(part 1 of 2)
# Autodesk Inventor assembly: Intake Full Assembly
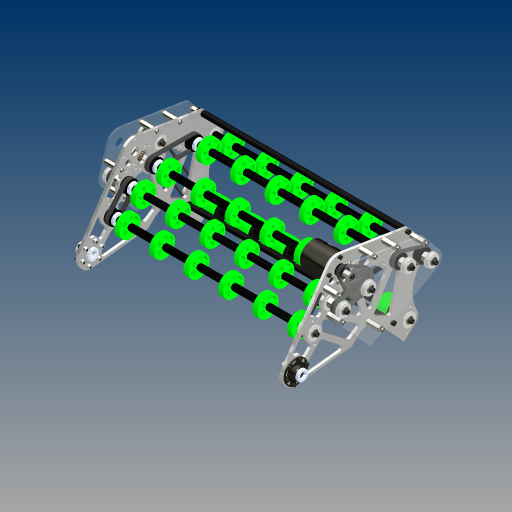
[picture p0: Inventor's stored thumbnail of the model, 512x512]
Saved by Autodesk Inventor 2024.3 (Build 283343000, 343)
## iProperties
Created: 2024-07-29
Part Number: Intake Full Assembly
Document SubType Name: Assembly
Designer: Kenji
Mass: 5624.47 g
Surface Area: 12461.9 cm^2
Volume: 2500.15 cm^3
Density: 2.24965 g/cm^3
Author: Kenji
## Documents named in this file (37)
- C:\Users\Kenji\Documents\GitHub\1622-2024-Summer-CAD-A-Thon\Intake\Intake Full Assembly.iam
- C:\Users\Kenji\Documents\GitHub\1622-2024-Summer-CAD-A-Thon\Intake\Intake Roller Plate.ipt
- C:\Users\Kenji\Documents\GitHub\1622-2024-Summer-CAD-A-Thon\COTS Library\Motion\Bearings\COTS_WCP-0783_1.125ODHexBearing.ipt
- C:\Users\Kenji\Documents\GitHub\1622-2024-Summer-CAD-A-Thon\Intake\Intake HexShaft 1.ipt
- C:\Users\Kenji\Documents\GitHub\1622-2024-Summer-CAD-A-Thon\COTS Library\Motion\Wheels\Compliant Wheels\2in compliant wheels\0.500in hex bore\COTS_am-3462_2indiameter_0.500inhexbore_durometer35A_CompliantWheel.ipt
- C:\Users\Kenji\Documents\GitHub\1622-2024-Summer-CAD-A-Thon\COTS Library\Motion\Wheels\Stealth Wheels\COTS_am-3155 2IN 500Hex Stealth Wheel.iam
- C:\Users\Kenji\Documents\GitHub\1622-2024-Summer-CAD-A-Thon\COTS Library\Structural Adapter\VersaHubs\COTS_217-2592_VersaHub.ipt
- C:\Users\Kenji\Documents\GitHub\1622-2024-Summer-CAD-A-Thon\Intake\Intake BeaterBar.ipt
- C:\Users\Kenji\Documents\GitHub\1622-2024-Summer-CAD-A-Thon\COTS Library\Fasteners\Bolts\Socket-Head\0.25-20\COTS_91251A539_Black-Oxide Alloy Steel Socket Head Screw (1).ipt
- C:\Users\Kenji\Documents\GitHub\1622-2024-Summer-CAD-A-Thon\COTS Library\Fasteners\Washers\COTS_90107A029_316 Stainless Steel Washer.ipt
- C:\Users\Kenji\Documents\GitHub\1622-2024-Summer-CAD-A-Thon\COTS Library\Fasteners\Shaft Collars\COTS_WCP-0799_0.5inchHexShaftCollar.ipt
- C:\Users\Kenji\Documents\GitHub\1622-2024-Summer-CAD-A-Thon\COTS Library\Motors\COTS_REV-21-1650-V1.1.ipt
- C:\Users\Kenji\Documents\GitHub\1622-2024-Summer-CAD-A-Thon\Intake\Intake Hex Shaft 3.ipt
- C:\Users\Kenji\Documents\GitHub\1622-2024-Summer-CAD-A-Thon\COTS Library\Motion\Pulleys\HTD5M\10mm Wide\COTW_HTD5M10mm12T_WCP-0076.ipt
- C:\Users\Kenji\Documents\GitHub\1622-2024-Summer-CAD-A-Thon\COTS Library\Motion\Pulleys\HTD5M\10mm Wide\COTS_HTD5M10mm36T_WCP-0990.ipt
- C:\Users\Kenji\Documents\GitHub\1622-2024-Summer-CAD-A-Thon\COTS Library\Motion\Gears\20DP gears\Aluminum\COTS_WCP-0706_30T.ipt
- C:\Users\Kenji\Documents\GitHub\1622-2024-Summer-CAD-A-Thon\COTS Library\Motion\Pulleys\HTD5M\10mm Wide\COTS_HTD5M10mm18T_WCP-0563.ipt
- C:\Users\Kenji\Documents\GitHub\1622-2024-Summer-CAD-A-Thon\Intake\INTK_002_HexShaft4.ipt
- C:\Users\Kenji\Documents\GitHub\1622-2024-Summer-CAD-A-Thon\Intake\INTK_003_HexShaft5.ipt
- C:\Users\Kenji\Documents\GitHub\1622-2024-Summer-CAD-A-Thon\Intake\INTK_001_PulleyCover.ipt
- C:\Users\Kenji\Documents\GitHub\1622-2024-Summer-CAD-A-Thon\Intake\INTK_004_HexShaft6.ipt
- C:\Users\Kenji\Documents\GitHub\1622-2024-Summer-CAD-A-Thon\Intake\INTK_005_Spacer5.ipt
- C:\Users\Kenji\Documents\GitHub\1622-2024-Summer-CAD-A-Thon\Intake\INTK_006_Spacer6.ipt
- C:\Users\Kenji\Documents\GitHub\1622-2024-Summer-CAD-A-Thon\COTS Library\Fasteners\Bolts\Socket-Head\10-32\COTS_91251A342_1-2in Long_Black-Oxide Alloy Steel Socket Head.ipt
- C:\Users\Kenji\Documents\GitHub\1622-2024-Summer-CAD-A-Thon\COTS Library\Fasteners\Washers\COTS_91860A047_Size10Washer.ipt
- C:\Users\Kenji\Documents\GitHub\1622-2024-Summer-CAD-A-Thon\COTS Library\Motion\Pulleys\HTD5M\10mm Wide\COTS_HTD5M10mm15T_WCP-1420.ipt
- C:\Users\Kenji\Documents\GitHub\1622-2024-Summer-CAD-A-Thon\Intake\INTK_007_Spacer7.ipt
- C:\Users\Kenji\Documents\GitHub\1622-2024-Summer-CAD-A-Thon\COTS Library\Fasteners\Bolts\Button-Head\10-32\COTS_92949A265_1-2in long Stainless Steel Button Head Screw.ipt
- C:\Users\Kenji\Documents\GitHub\1622-2024-Summer-CAD-A-Thon\COTS Library\Fasteners\Bolts\Socket-Head\8-32\COTS_91251A196_Black-Oxide Alloy Steel Socket Head Screw_5-8in.ipt
- C:\Users\Kenji\Documents\GitHub\1622-2024-Summer-CAD-A-Thon\COTS Library\Fasteners\Nuts\COTS_90631A009_8-32_Low-Strength Steel Nylon-Insert Locknut.ipt
- C:\Users\Kenji\Documents\GitHub\1622-2024-Summer-CAD-A-Thon\Intake\INTK_009_Belt1.ipt
- C:\Users\Kenji\Documents\GitHub\1622-2024-Summer-CAD-A-Thon\Intake\INtk_010_Belt2.ipt
- C:\Users\Kenji\Documents\GitHub\1622-2024-Summer-CAD-A-Thon\Intake\INTK_011_Belt3.ipt
- C:\Users\Kenji\Documents\GitHub\1622-2024-Summer-CAD-A-Thon\Intake\INTK_012_Belt4.ipt
- C:\Users\Kenji\Documents\GitHub\1622-2024-Summer-CAD-A-Thon\Intake\INTK_013_Belt5.ipt
- C:\Users\Kenji\Documents\GitHub\1622-2024-Summer-CAD-A-Thon\Intake\INTK_014_Belt6.ipt
- C:\Users\Kenji\Documents\GitHub\1622-2024-Summer-CAD-A-Thon\Intake\INTK_015_Spacer8.ipt
## Components (226 placed, 36 different names)
1. Intake Roller Plate:1 — Mate:293, Mate:294, Mate:295, Mate:296, Mate:297, Mate:298, Mate:299, Mate:302, Mate:303, Mate:304, Mate:306, Mate:307, Mate:308, Mate:310, Mate:311, Mate:312, Mate:313, Mate:315, Mate:316, Mate:317, Mate:318, Mate:319, Mate:320, Mate:321, Mate:481, Mate:520, Mate:521, Mate:525, Mate:527, Mate:553, Mate:555, Mate:577, Mate:578, Mate:579, Mate:580, Mate:581, Mate:584, Mate:585, Mate:586, Mate:587, Mate:588, Mate:664, Mate:665, Mate:666, Mate:667, Mate:668, Mate:669, Mate:670, Mate:674, Mate:705, Mate:706, Mate:733, Mate:736, Mate:749, Mate:786
2. Intake Roller Plate:2 — Mate:270, Mate:272, Mate:273, Mate:275, Mate:276, Mate:277, Mate:278, Mate:279, Mate:280, Mate:281, Mate:282, Mate:283, Mate:284, Mate:285, Mate:286, Mate:287, Mate:290, Mate:291, Mate:292, Mate:300, Mate:301, Mate:347, Mate:348, Mate:611, Mate:612, Mate:613, Mate:614, Mate:615, Mate:617, Mate:618, Mate:619, Mate:620, Mate:621, Mate:647, Mate:649, Mate:651, Mate:653, Mate:655, Mate:657, Mate:695, Mate:774, Mate:776, Mate:782, Mate:783
3. COTS_WCP-0783_1.125ODHexBearing:1 — Mate:25, Mate:276, Mate:283, Mate:329, Mate:340, Flush:10, Mate:355, Mate:428
4. COTS_WCP-0783_1.125ODHexBearing:2 — Mate:26, Mate:277, Mate:278, Mate:334, Mate:379, Mate:406, Mate:501
5. COTS_WCP-0783_1.125ODHexBearing:3 — Mate:272, Mate:280, Mate:332, Mate:458, Mate:482, Mate:541
6. COTS_WCP-0783_1.125ODHexBearing:4 — Mate:233, Mate:275, Mate:282, Mate:330, Mate:423, Mate:427, Mate:430, Mate:529
7. COTS_WCP-0783_1.125ODHexBearing:5 — Mate:270, Mate:271, Mate:279, Mate:333, Mate:479, Mate:480
8. COTS_WCP-0783_1.125ODHexBearing:6 — Mate:273, Mate:274, Mate:281, Mate:331, Mate:372, Mate:374, Mate:405, Mate:467, Mate:468, Mate:469
9. COTS_WCP-0783_1.125ODHexBearing:7 — Mate:319, Mate:320, Mate:326, Mate:441, Mate:455, Mate:456, Mate:485
10. COTS_WCP-0783_1.125ODHexBearing:8 — Mate:315, Mate:316, Mate:324, Mate:434, Mate:435, Mate:508, Mate:534
11. COTS_WCP-0783_1.125ODHexBearing:9 — Mate:317, Mate:318, Mate:370, Mate:371, Mate:407, Mate:442, Mate:463, Mate:464
12. COTS_WCP-0783_1.125ODHexBearing:10 — Mate:25, Mate:294, Mate:295, Mate:323, Mate:425, Mate:432, Mate:433, Mate:448
13. COTS_WCP-0783_1.125ODHexBearing:11 — Mate:26, Mate:132, Mate:144, Mate:293, Mate:321, Mate:328, Mate:402, Flush:17, Mate:403
14. COTS_WCP-0783_1.125ODHexBearing:12 — Mate:33, Mate:313, Mate:327, Mate:481, Mate:483, Mate:484
15. COTS_217-2592_VersaHub:2 — Mate:262, Mate:263, Mate:302, Mate:303, Mate:304, Mate:305, Mate:622, Mate:623, Mate:624, Mate:625, Mate:626, Mate:627, Mate:628, Mate:629, Mate:630, Mate:631, Mate:632, Mate:633
16. COTS_217-2592_VersaHub:3 — Mate:266, Mate:267, Mate:284, Mate:285, Mate:286, Mate:634, Mate:635, Mate:636, Mate:637, Mate:638, Mate:639, Mate:640, Mate:641, Mate:642, Mate:643, Mate:644, Mate:645
17. Intake BeaterBar:1 — Mate:251, Mate:297, Mate:298
18. Intake BeaterBar:2 — Mate:253, Mate:289, Mate:290, Mate:291, Mate:312
19. COTS_91251A539_Black-Oxide Alloy Steel Socket Head Screw (1):1 — Mate:212, Mate:213
20. COTS_91251A539_Black-Oxide Alloy Steel Socket Head Screw (1):2 — Mate:253, Mate:296
21. COTS_91251A539_Black-Oxide Alloy Steel Socket Head Screw (1):3 — Mate:375, Mate:408, Mate:409
22. COTS_91251A539_Black-Oxide Alloy Steel Socket Head Screw (1):4 — Mate:204, Mate:322
23. COTS_91251A539_Black-Oxide Alloy Steel Socket Head Screw (1):5 — Mate:195, Mate:196, Mate:500
24. COTS_91251A539_Black-Oxide Alloy Steel Socket Head Screw (1):6 — Mate:210, Mate:211, Mate:512
25. COTS_91251A539_Black-Oxide Alloy Steel Socket Head Screw (1):7 — Mate:189, Mate:190
26. COTS_91251A539_Black-Oxide Alloy Steel Socket Head Screw (1):8 — Mate:193, Mate:194, Mate:502
27. COTS_91251A539_Black-Oxide Alloy Steel Socket Head Screw (1):9 — Mate:251, Mate:300, Mate:301
28. COTS_91251A539_Black-Oxide Alloy Steel Socket Head Screw (1):10 — Mate:289, Mate:292
29. COTS_91251A539_Black-Oxide Alloy Steel Socket Head Screw (1):11 — Mate:216, Mate:217
30. COTS_91251A539_Black-Oxide Alloy Steel Socket Head Screw (1):12 — Mate:218, Mate:219
31. COTS_91251A539_Black-Oxide Alloy Steel Socket Head Screw (1):13 — Mate:299, Mate:307
32. COTS_91251A539_Black-Oxide Alloy Steel Socket Head Screw (1):14 — Mate:191, Mate:192, Mate:457, Mate:459, Mate:504
33. COTS_91251A539_Black-Oxide Alloy Steel Socket Head Screw (1):15 — Mate:187, Mate:233, Mate:426, Mate:506
34. COTS_91251A539_Black-Oxide Alloy Steel Socket Head Screw (1):16 — Mate:185, Mate:186
35. COTS_90107A029_316 Stainless Steel Washer:1 — Mate:212, Mate:213, Mate:326, Mate:499, Mate:510
36. COTS_90107A029_316 Stainless Steel Washer:2 — Mate:408, Mate:409, Mate:414
37. COTS_90107A029_316 Stainless Steel Washer:3 — Mate:193, Mate:194, Mate:271, Mate:333, Mate:496
38. COTS_90107A029_316 Stainless Steel Washer:4 — Mate:216, Mate:217, Mate:324, Mate:454, Mate:472
39. COTS_90107A029_316 Stainless Steel Washer:5 — Mate:187, Mate:330, Mate:426, Mate:476
40. COTS_90107A029_316 Stainless Steel Washer:6 — Mate:210, Mate:211, Mate:327, Mate:498
41. COTS_90107A029_316 Stainless Steel Washer:7 — Mate:204, Mate:322, Mate:328, Mate:403
42. COTS_90107A029_316 Stainless Steel Washer:8 — Mate:185, Mate:186, Mate:329, Mate:355
43. COTS_90107A029_316 Stainless Steel Washer:9 — Mate:218, Mate:219, Mate:323, Mate:448
44. COTS_90107A029_316 Stainless Steel Washer:10 — Mate:189, Mate:190, Mate:274, Mate:331, Mate:390
45. COTS_90107A029_316 Stainless Steel Washer:11 — Mate:195, Mate:196, Mate:334, Mate:392
46. COTS_90107A029_316 Stainless Steel Washer:12 — Mate:191, Mate:192, Mate:332, Mate:497
47. COTS_WCP-0799_0.5inchHexShaftCollar:1 — Mate:305, Mate:306
48. COTS_WCP-0799_0.5inchHexShaftCollar:2 — Mate:266, Mate:267, Mate:288
49. COTS_WCP-0799_0.5inchHexShaftCollar:3 — Mate:262, Mate:263
50. COTS_WCP-0799_0.5inchHexShaftCollar:4 — Mate:287, Mate:288
51. COTS_REV-21-1650-V1.1:2 — Mate:308, Mate:310, Mate:311, Flush:8, Mate:369, Mate:514, Flush:30, Mate:515, Mate:707, Mate:708
52. Intake HexShaft 1:6 — Mate:340, Flush:10
53. COTS_WCP-0783_1.125ODHexBearing:13 — Mate:347, Mate:348, Mate:373, Mate:376, Mate:404
54. Intake Hex Shaft 3:1 — Flush:8, Mate:375, Mate:407, Mate:410
55. COTS_WCP-0783_1.125ODHexBearing:14 — Mate:410, Mate:414, Mate:676, Mate:678, Mate:726, Mate:727
56. COTW_HTD5M10mm12T_WCP-0076:1 — Mate:369, Flush:14, Mate:680
57. COTS_HTD5M10mm36T_WCP-0990:1 — Mate:370, Mate:371, Flush:14, Mate:535, Mate:536
58. COTS_WCP-0706_30T:1 — Mate:372, Mate:374, Mate:530, Mate:531
59. COTS_WCP-0706_30T:2 — Mate:373, Mate:376, Mate:377, Mate:378
60. COTS_HTD5M10mm18T_WCP-0563:1 — Mate:377, Mate:378, Mate:389, Flush:29, Mate:704
61. COTS_HTD5M10mm18T_WCP-0563:2 — Mate:379, Flush:29
62. COTS_WCP-0783_1.125ODHexBearing:15 — Mate:390, Mate:405, Mate:682, Mate:777
63. COTS_WCP-0783_1.125ODHexBearing:16 — Mate:392, Mate:406, Flush:19
64. COTS_WCP-0783_1.125ODHexBearing:17 — Mate:389, Mate:393, Flush:16, Mate:404, Mate:703
65. INTK_002_HexShaft4:2 — Mate:393, Flush:16, Mate:398, Mate:399, Mate:400, Mate:401
66. COTS_91251A539_Black-Oxide Alloy Steel Socket Head Screw (1):17 — Mate:394, Mate:395, Mate:400
67. COTS_91251A539_Black-Oxide Alloy Steel Socket Head Screw (1):18 — Mate:396, Mate:397
68. COTS_90107A029_316 Stainless Steel Washer:13 — Mate:394, Mate:395, Mate:401
69. COTS_90107A029_316 Stainless Steel Washer:14 — Mate:396, Mate:397, Mate:398, Mate:399
70. INTK_003_HexShaft5:1 — Mate:402, Flush:17, Flush:19
71. INTK_001_PulleyCover:1 — Mate:723, Mate:724, Mate:725, Mate:726, Mate:727, Mate:729, Mate:730, Mate:731, Mate:732, Mate:734, Mate:735, Mate:737, Mate:739, Mate:740, Mate:742, Mate:743, Mate:744, Mate:746, Mate:747, Mate:748, Mate:787
72. INTK_001_PulleyCover:2 — Mate:750, Mate:751, Mate:752, Mate:753, Mate:754, Mate:756, Mate:757, Mate:758, Mate:760, Mate:761, Mate:762, Mate:763, Mate:764, Mate:765, Mate:766, Mate:767, Mate:769, Mate:770, Mate:771, Mate:772, Mate:773, Mate:774, Mate:777, Mate:778, Mate:779, Mate:780, Mate:781
73. COTS_HTD5M10mm18T_WCP-0563:4 — Mate:455, Mate:456, Mate:461, Mate:462, Mate:692
74. COTS_HTD5M10mm18T_WCP-0563:5 — Mate:425, Flush:21, Mate:429, Mate:784
75. COTS_HTD5M10mm18T_WCP-0563:6 — Mate:423, Flush:21, Mate:427, Mate:431
76. COTS_HTD5M10mm18T_WCP-0563:9 — Mate:468, Mate:469, Mate:470
77. COTS_HTD5M10mm18T_WCP-0563:11 — Mate:479, Mate:480, Mate:503, Mate:701
78. COTS_HTD5M10mm18T_WCP-0563:12 — Mate:457, Mate:458, Mate:460
79. COTS_HTD5M10mm18T_WCP-0563:13 — Mate:482, Mate:540, Mate:541
80. COTS_HTD5M10mm18T_WCP-0563:14 — Mate:463, Mate:464, Mate:465, Mate:466
81. COTS_HTD5M10mm18T_WCP-0563:15 — Mate:483, Mate:484, Flush:26, Mate:698
82. COTS_HTD5M10mm18T_WCP-0563:16 — Mate:434, Mate:435, Mate:438, Mate:439, Mate:785
83. COTS_HTD5M10mm18T_WCP-0563:17 — Mate:485, Flush:26, Mate:511
84. COTS_HTD5M10mm18T_WCP-0563:18 — Mate:432, Mate:433, Mate:436, Mate:437
85. COTS_WCP-0799_0.5inchHexShaftCollar:5 — Mate:428, Mate:429, Mate:688
86. COTS_WCP-0799_0.5inchHexShaftCollar:6 — Mate:430, Mate:431, Mate:687
87. COTS_WCP-0799_0.5inchHexShaftCollar:7 — Mate:436, Mate:437, Mate:440, Mate:444, Mate:685
88. COTS_WCP-0799_0.5inchHexShaftCollar:8 — Mate:438, Mate:439, Mate:443, Mate:445, Mate:684
89. INTK_004_HexShaft6:1 — Mate:454, Mate:710
90. COTS_WCP-0783_1.125ODHexBearing:19 — Mate:472, Mate:537, Mate:539, Mate:675, Mate:709, Mate:724, Mate:725
91. COTS_WCP-0799_0.5inchHexShaftCollar:9 — Mate:461, Mate:462, Mate:691
92. COTS_WCP-0799_0.5inchHexShaftCollar:10 — Mate:459, Mate:460, Mate:693
93. COTS_WCP-0799_0.5inchHexShaftCollar:11 — Mate:465, Mate:466, Mate:690
94. COTS_WCP-0799_0.5inchHexShaftCollar:12 — Mate:467, Mate:470, Mate:694
95. COTS_WCP-0783_1.125ODHexBearing:20 — Mate:476, Mate:681, Mate:778
96. INTK_004_HexShaft6:2 — Mate:711, Flush:32
97. INTK_004_HexShaft6:3 — Flush:31, Mate:713
98. COTS_WCP-0783_1.125ODHexBearing:21 — Mate:498, Mate:513, Mate:730, Mate:787
99. COTS_WCP-0783_1.125ODHexBearing:22 — Mate:499, Flush:31, Mate:729, Mate:731
100. COTS_WCP-0783_1.125ODHexBearing:23 — Mate:497, Mate:505, Mate:781
101. COTS_WCP-0783_1.125ODHexBearing:24 — Mate:496, Mate:779, Mate:780, Flush:32
102. INTK_005_Spacer5:1 — Mate:506, Mate:529, Mate:532, Mate:533, Mate:713
103. INTK_005_Spacer5:2 — Mate:504, Mate:505, Mate:540, Mate:700, Mate:711
104. INTK_005_Spacer5:3 — Mate:500, Mate:501, Mate:702
105. INTK_005_Spacer5:4 — Mate:502, Mate:503, Mate:699, Mate:710
106. INTK_005_Spacer5:5 — Mate:508, Mate:534, Mate:538, Mate:709
107. INTK_005_Spacer5:6 — Mate:510, Mate:511, Mate:696
108. INTK_005_Spacer5:7 — Mate:512, Mate:513, Mate:697
109. INTK_006_Spacer6:1 — Mate:514, Flush:30, Mate:518, Mate:679, Mate:723
110. COTS_91251A342_1-2in Long_Black-Oxide Alloy Steel Socket Head:1 — Mate:520, Mate:527
111. COTS_91251A342_1-2in Long_Black-Oxide Alloy Steel Socket Head:3 — Mate:515, Mate:516, Mate:517
112. COTS_91251A342_1-2in Long_Black-Oxide Alloy Steel Socket Head:6 — Mate:521, Mate:525
113. COTS_91860A047_Size10Washer:1 — Mate:516, Mate:517, Mate:518
114. COTS_HTD5M10mm15T_WCP-1420:1 — Mate:532, Mate:533, Mate:683, Mate:714
115. COTS_HTD5M10mm15T_WCP-1420:2 — Mate:530, Mate:531
116. COTS_HTD5M10mm15T_WCP-1420:3 — Mate:537, Mate:538, Mate:539
117. COTS_HTD5M10mm15T_WCP-1420:4 — Mate:535, Mate:536, Mate:677
118. INTK_007_Spacer7:1 — Mate:553, Mate:718, Mate:747
119. INTK_007_Spacer7:2 — Mate:762, Mate:765
120. INTK_007_Spacer7:3 — Mate:766, Mate:767, Mate:768
121. INTK_007_Spacer7:4 — Mate:715, Mate:741, Mate:742
122. INTK_007_Spacer7:5 — Mate:750, Mate:753, Mate:775
123. INTK_007_Spacer7:7 — Mate:759, Mate:761, Mate:776
124. INTK_007_Spacer7:8 — Mate:555, Mate:720, Mate:745
125. INTK_007_Spacer7:11 — Mate:770, Mate:771
126. INTK_007_Spacer7:12 — Mate:755, Mate:756
127. INTK_007_Spacer7:14 — Mate:721, Mate:732, Mate:733
128. INTK_007_Spacer7:15 — Mate:717, Mate:722, Mate:735, Mate:736
129. INTK_007_Spacer7:16 — Mate:716, Mate:738, Mate:739
130. COTS_92949A265_1-2in long Stainless Steel Button Head Screw:1 — Mate:768, Mate:769
131. COTS_92949A265_1-2in long Stainless Steel Button Head Screw:2 — Mate:758, Mate:759, Mate:760
132. COTS_92949A265_1-2in long Stainless Steel Button Head Screw:3 — Mate:754, Mate:755, Mate:757
133. COTS_92949A265_1-2in long Stainless Steel Button Head Screw:4 — Mate:763, Mate:764
134. COTS_92949A265_1-2in long Stainless Steel Button Head Screw:5 — Mate:751, Mate:752
135. COTS_92949A265_1-2in long Stainless Steel Button Head Screw:6 — Mate:577, Mate:586, Mate:741
136. COTS_92949A265_1-2in long Stainless Steel Button Head Screw:7 — Mate:715, Mate:743, Mate:744
137. COTS_92949A265_1-2in long Stainless Steel Button Head Screw:8 — Mate:579, Mate:588
138. COTS_92949A265_1-2in long Stainless Steel Button Head Screw:11 — Mate:611, Mate:621
139. COTS_92949A265_1-2in long Stainless Steel Button Head Screw:12 — Mate:772, Mate:773
140. COTS_92949A265_1-2in long Stainless Steel Button Head Screw:13 — Mate:782, Mate:783
141. COTS_92949A265_1-2in long Stainless Steel Button Head Screw:14 — Mate:721, Mate:734
142. COTS_92949A265_1-2in long Stainless Steel Button Head Screw:15 — Mate:717, Mate:722, Mate:737
143. COTS_92949A265_1-2in long Stainless Steel Button Head Screw:16 — Mate:716, Mate:740
144. COTS_92949A265_1-2in long Stainless Steel Button Head Screw:17 — Mate:749, Mate:786
145. COTS_92949A265_1-2in long Stainless Steel Button Head Screw:18 — Mate:718, Mate:748
146. COTS_92949A265_1-2in long Stainless Steel Button Head Screw:19 — Mate:580, Mate:585, Mate:738
147. COTS_92949A265_1-2in long Stainless Steel Button Head Screw:20 — Mate:578, Mate:587, Mate:745
148. COTS_92949A265_1-2in long Stainless Steel Button Head Screw:21 — Mate:581, Mate:584
149. COTS_92949A265_1-2in long Stainless Steel Button Head Screw:22 — Mate:615, Mate:617
150. COTS_92949A265_1-2in long Stainless Steel Button Head Screw:23 — Mate:614, Mate:618
151. COTS_92949A265_1-2in long Stainless Steel Button Head Screw:24 — Mate:720, Mate:746
152. COTS_92949A265_1-2in long Stainless Steel Button Head Screw:25 — Mate:612, Mate:620
153. COTS_92949A265_1-2in long Stainless Steel Button Head Screw:27 — Mate:613, Mate:619, Mate:775
154. COTS_91251A196_Black-Oxide Alloy Steel Socket Head Screw_5-8in:1 — Mate:623, Mate:633, Mate:663
155. COTS_91251A196_Black-Oxide Alloy Steel Socket Head Screw_5-8in:2 — Mate:624, Mate:631, Mate:659
156. COTS_91251A196_Black-Oxide Alloy Steel Socket Head Screw_5-8in:3 — Mate:622, Mate:632, Mate:658
157. COTS_91251A196_Black-Oxide Alloy Steel Socket Head Screw_5-8in:4 — Mate:626, Mate:628, Mate:660
158. COTS_91251A196_Black-Oxide Alloy Steel Socket Head Screw_5-8in:5 — Mate:638, Mate:644, Mate:654
159. COTS_91251A196_Black-Oxide Alloy Steel Socket Head Screw_5-8in:6 — Mate:627, Mate:629, Mate:661
160. COTS_91251A196_Black-Oxide Alloy Steel Socket Head Screw_5-8in:7 — Mate:635, Mate:641, Mate:650
161. COTS_91251A196_Black-Oxide Alloy Steel Socket Head Screw_5-8in:8 — Mate:639, Mate:643, Mate:648
162. COTS_91251A196_Black-Oxide Alloy Steel Socket Head Screw_5-8in:9 — Mate:637, Mate:645, Mate:656
163. COTS_91251A196_Black-Oxide Alloy Steel Socket Head Screw_5-8in:10 — Mate:636, Mate:642, Mate:646
164. COTS_91251A196_Black-Oxide Alloy Steel Socket Head Screw_5-8in:11 — Mate:625, Mate:630, Mate:662
165. COTS_91251A196_Black-Oxide Alloy Steel Socket Head Screw_5-8in:12 — Mate:634, Mate:640, Mate:652
166. COTS_90631A009_8-32_Low-Strength Steel Nylon-Insert Locknut:1 — Mate:648, Mate:649
167. COTS_90631A009_8-32_Low-Strength Steel Nylon-Insert Locknut:2 — Mate:662, Mate:669
168. COTS_90631A009_8-32_Low-Strength Steel Nylon-Insert Locknut:3 — Mate:663, Mate:664
169. COTS_90631A009_8-32_Low-Strength Steel Nylon-Insert Locknut:4 — Mate:652, Mate:653
170. COTS_90631A009_8-32_Low-Strength Steel Nylon-Insert Locknut:5 — Mate:658, Mate:665
171. COTS_90631A009_8-32_Low-Strength Steel Nylon-Insert Locknut:6 — Mate:661, Mate:668
172. COTS_90631A009_8-32_Low-Strength Steel Nylon-Insert Locknut:7 — Mate:656, Mate:657
173. COTS_90631A009_8-32_Low-Strength Steel Nylon-Insert Locknut:8 — Mate:654, Mate:655
174. COTS_90631A009_8-32_Low-Strength Steel Nylon-Insert Locknut:9 — Mate:659, Mate:666
175. COTS_90631A009_8-32_Low-Strength Steel Nylon-Insert Locknut:10 — Mate:660, Mate:667
176. COTS_90631A009_8-32_Low-Strength Steel Nylon-Insert Locknut:11 — Mate:646, Mate:647
177. COTS_90631A009_8-32_Low-Strength Steel Nylon-Insert Locknut:12 — Mate:650, Mate:651
178. COTS_92949A265_1-2in long Stainless Steel Button Head Screw:28 — Mate:670, Mate:674
179. COTS_92949A265_1-2in long Stainless Steel Button Head Screw:29 — Mate:705, Mate:706
180. INTK_009_Belt1:1 — Mate:678, Mate:679, Mate:680
181. INtk_010_Belt2:1 — Mate:675, Mate:676, Mate:677
182. INtk_010_Belt2:2 — Mate:681, Mate:682, Mate:683, Mate:714
183. INTK_011_Belt3:1 — Mate:684, Mate:685, Mate:785
184. INTK_011_Belt3:2 — Mate:687, Mate:688, Mate:784
185. INTK_012_Belt4:1 — Mate:690, Mate:691, Mate:692
186. INTK_012_Belt4:2 — Mate:693, Mate:694, Mate:695
187. INTK_013_Belt5:1 — Mate:696, Mate:697, Mate:698
188. INTK_013_Belt5:2 — Mate:699, Mate:700, Mate:701
189. INTK_014_Belt6:1 — Mate:702, Mate:703, Mate:704
190. INTK_015_Spacer8:1 — Mate:707, Mate:708
191. COTS_am-3155 2IN 500Hex Stealth Wheel:7 [sub-assembly] — Mate:132, Mate:144
192. COTS_am-3155 2IN 500Hex Stealth Wheel:8 [sub-assembly]
193. COTS_am-3155 2IN 500Hex Stealth Wheel:9 [sub-assembly]
194. COTS_am-3155 2IN 500Hex Stealth Wheel:10 [sub-assembly]
195. COTS_am-3155 2IN 500Hex Stealth Wheel:11 [sub-assembly]
196. COTS_am-3155 2IN 500Hex Stealth Wheel:12 [sub-assembly]
197. COTS_am-3462_2indiameter_0.500inhexbore_durometer35A_CompliantWheel:53 — Mate:440, Mate:444
198. COTS_am-3462_2indiameter_0.500inhexbore_durometer35A_CompliantWheel:66 — Mate:443, Mate:445, Flush:22
199. COTS_am-3462_2indiameter_0.500inhexbore_durometer35A_CompliantWheel:40 — Mate:442, Flush:22, Flush:23
200. COTS_am-3462_2indiameter_0.500inhexbore_durometer35A_CompliantWheel:25 — Mate:441, Flush:23, Flush:24
201. COTS_am-3462_2indiameter_0.500inhexbore_durometer35A_CompliantWheel:24 — Mate:33, Flush:24
202. COTS_am-3462_2indiameter_0.500inhexbore_durometer35A_CompliantWheel:67
203. COTS_am-3462_2indiameter_0.500inhexbore_durometer35A_CompliantWheel:68
204. COTS_am-3462_2indiameter_0.500inhexbore_durometer35A_CompliantWheel:69
205. COTS_am-3462_2indiameter_0.500inhexbore_durometer35A_CompliantWheel:70
206. COTS_am-3462_2indiameter_0.500inhexbore_durometer35A_CompliantWheel:71
207. COTS_am-3462_2indiameter_0.500inhexbore_durometer35A_CompliantWheel:72
208. COTS_am-3462_2indiameter_0.500inhexbore_durometer35A_CompliantWheel:73
209. COTS_am-3462_2indiameter_0.500inhexbore_durometer35A_CompliantWheel:74
210. COTS_am-3462_2indiameter_0.500inhexbore_durometer35A_CompliantWheel:75
211. COTS_am-3462_2indiameter_0.500inhexbore_durometer35A_CompliantWheel:76
212. COTS_am-3462_2indiameter_0.500inhexbore_durometer35A_CompliantWheel:77
213. COTS_am-3462_2indiameter_0.500inhexbore_durometer35A_CompliantWheel:78
214. COTS_am-3462_2indiameter_0.500inhexbore_durometer35A_CompliantWheel:79
215. COTS_am-3462_2indiameter_0.500inhexbore_durometer35A_CompliantWheel:80
216. COTS_am-3462_2indiameter_0.500inhexbore_durometer35A_CompliantWheel:81
217. COTS_am-3462_2indiameter_0.500inhexbore_durometer35A_CompliantWheel:82
218. COTS_am-3462_2indiameter_0.500inhexbore_durometer35A_CompliantWheel:83
219. COTS_am-3462_2indiameter_0.500inhexbore_durometer35A_CompliantWheel:84
220. COTS_am-3462_2indiameter_0.500inhexbore_durometer35A_CompliantWheel:85
221. COTS_am-3462_2indiameter_0.500inhexbore_durometer35A_CompliantWheel:86
222. COTS_am-3462_2indiameter_0.500inhexbore_durometer35A_CompliantWheel:87
223. COTS_am-3462_2indiameter_0.500inhexbore_durometer35A_CompliantWheel:88
224. COTS_am-3462_2indiameter_0.500inhexbore_durometer35A_CompliantWheel:89
225. COTS_am-3462_2indiameter_0.500inhexbore_durometer35A_CompliantWheel:90
226. COTS_am-3462_2indiameter_0.500inhexbore_durometer35A_CompliantWheel:91
## Component patterns: (6 elements, first: COTS_am-3155 2IN 500Hex Stealth Wheel:7), (6 elements, first: COTS_am-3462_2indiameter_0.500inhexbore_durometer35A_CompliantWheel:53 + COTS_am-3462_2indiameter_0.500inhexbore_durometer35A_CompliantWheel:66 + COTS_am-3462_2indiameter_0.500inhexbore_durometer35A_CompliantWheel:40 + COTS_am-3462_2indiameter_0.500inhexbore_durometer35A_CompliantWheel:25 + COTS_am-3462_2indiameter_0.500inhexbore_durometer35A_CompliantWheel:24)
## Relationships (413: Mate 398, Flush 15)
- Mate:25: COTS_WCP-0783_1.125ODHexBearing:1 ↔ COTS_WCP-0783_1.125ODHexBearing:10
- Mate:26: COTS_WCP-0783_1.125ODHexBearing:2 ↔ COTS_WCP-0783_1.125ODHexBearing:11
- Mate:33: COTS_WCP-0783_1.125ODHexBearing:12 ↔ COTS_am-3462_2indiameter_0.500inhexbore_durometer35A_CompliantWheel:24
- Mate:132 (27.94 mm): COTS_WCP-0783_1.125ODHexBearing:11 ↔ COTS_am-3155 2IN 500Hex Stealth Wheel:7
- Mate:144: COTS_WCP-0783_1.125ODHexBearing:11 ↔ COTS_am-3155 2IN 500Hex Stealth Wheel:7
- Mate:185: COTS_91251A539_Black-Oxide Alloy Steel Socket Head Screw (1):16 ↔ COTS_90107A029_316 Stainless Steel Washer:8
- Mate:186: COTS_91251A539_Black-Oxide Alloy Steel Socket Head Screw (1):16 ↔ COTS_90107A029_316 Stainless Steel Washer:8
- Mate:187: COTS_91251A539_Black-Oxide Alloy Steel Socket Head Screw (1):15 ↔ COTS_90107A029_316 Stainless Steel Washer:5
- Mate:189: COTS_91251A539_Black-Oxide Alloy Steel Socket Head Screw (1):7 ↔ COTS_90107A029_316 Stainless Steel Washer:10
- Mate:190: COTS_91251A539_Black-Oxide Alloy Steel Socket Head Screw (1):7 ↔ COTS_90107A029_316 Stainless Steel Washer:10
- Mate:191: COTS_91251A539_Black-Oxide Alloy Steel Socket Head Screw (1):14 ↔ COTS_90107A029_316 Stainless Steel Washer:12
- Mate:192: COTS_91251A539_Black-Oxide Alloy Steel Socket Head Screw (1):14 ↔ COTS_90107A029_316 Stainless Steel Washer:12
- Mate:193: COTS_91251A539_Black-Oxide Alloy Steel Socket Head Screw (1):8 ↔ COTS_90107A029_316 Stainless Steel Washer:3
- Mate:194: COTS_91251A539_Black-Oxide Alloy Steel Socket Head Screw (1):8 ↔ COTS_90107A029_316 Stainless Steel Washer:3
- Mate:195: COTS_91251A539_Black-Oxide Alloy Steel Socket Head Screw (1):5 ↔ COTS_90107A029_316 Stainless Steel Washer:11
- Mate:196: COTS_91251A539_Black-Oxide Alloy Steel Socket Head Screw (1):5 ↔ COTS_90107A029_316 Stainless Steel Washer:11
- Mate:204: COTS_91251A539_Black-Oxide Alloy Steel Socket Head Screw (1):4 ↔ COTS_90107A029_316 Stainless Steel Washer:7
- Mate:210: COTS_91251A539_Black-Oxide Alloy Steel Socket Head Screw (1):6 ↔ COTS_90107A029_316 Stainless Steel Washer:6
- Mate:211: COTS_91251A539_Black-Oxide Alloy Steel Socket Head Screw (1):6 ↔ COTS_90107A029_316 Stainless Steel Washer:6
- Mate:212: COTS_91251A539_Black-Oxide Alloy Steel Socket Head Screw (1):1 ↔ COTS_90107A029_316 Stainless Steel Washer:1
- Mate:213: COTS_91251A539_Black-Oxide Alloy Steel Socket Head Screw (1):1 ↔ COTS_90107A029_316 Stainless Steel Washer:1
- Mate:216: COTS_91251A539_Black-Oxide Alloy Steel Socket Head Screw (1):11 ↔ COTS_90107A029_316 Stainless Steel Washer:4
- Mate:217: COTS_91251A539_Black-Oxide Alloy Steel Socket Head Screw (1):11 ↔ COTS_90107A029_316 Stainless Steel Washer:4
- Mate:218: COTS_91251A539_Black-Oxide Alloy Steel Socket Head Screw (1):12 ↔ COTS_90107A029_316 Stainless Steel Washer:9
- Mate:219: COTS_91251A539_Black-Oxide Alloy Steel Socket Head Screw (1):12 ↔ COTS_90107A029_316 Stainless Steel Washer:9
- Mate:233: COTS_WCP-0783_1.125ODHexBearing:4 ↔ COTS_91251A539_Black-Oxide Alloy Steel Socket Head Screw (1):15
- Mate:251: Intake BeaterBar:1 ↔ COTS_91251A539_Black-Oxide Alloy Steel Socket Head Screw (1):9
- Mate:253: Intake BeaterBar:2 ↔ COTS_91251A539_Black-Oxide Alloy Steel Socket Head Screw (1):2
- Mate:262: COTS_217-2592_VersaHub:2 ↔ COTS_WCP-0799_0.5inchHexShaftCollar:3
- Mate:263: COTS_217-2592_VersaHub:2 ↔ COTS_WCP-0799_0.5inchHexShaftCollar:3
- Mate:266: COTS_217-2592_VersaHub:3 ↔ COTS_WCP-0799_0.5inchHexShaftCollar:2
- Mate:267: COTS_217-2592_VersaHub:3 ↔ COTS_WCP-0799_0.5inchHexShaftCollar:2
- Mate:270: Intake Roller Plate:2 ↔ COTS_WCP-0783_1.125ODHexBearing:5
- Mate:271: COTS_WCP-0783_1.125ODHexBearing:5 ↔ COTS_90107A029_316 Stainless Steel Washer:3
- Mate:272: Intake Roller Plate:2 ↔ COTS_WCP-0783_1.125ODHexBearing:3
- Mate:273: Intake Roller Plate:2 ↔ COTS_WCP-0783_1.125ODHexBearing:6
- Mate:274: COTS_WCP-0783_1.125ODHexBearing:6 ↔ COTS_90107A029_316 Stainless Steel Washer:10
- Mate:275: Intake Roller Plate:2 ↔ COTS_WCP-0783_1.125ODHexBearing:4
- Mate:276: Intake Roller Plate:2 ↔ COTS_WCP-0783_1.125ODHexBearing:1
- Mate:277: Intake Roller Plate:2 ↔ COTS_WCP-0783_1.125ODHexBearing:2
- Mate:278: Intake Roller Plate:2 ↔ COTS_WCP-0783_1.125ODHexBearing:2
- Mate:279: Intake Roller Plate:2 ↔ COTS_WCP-0783_1.125ODHexBearing:5
- Mate:280: Intake Roller Plate:2 ↔ COTS_WCP-0783_1.125ODHexBearing:3
- Mate:281: Intake Roller Plate:2 ↔ COTS_WCP-0783_1.125ODHexBearing:6
- Mate:282: Intake Roller Plate:2 ↔ COTS_WCP-0783_1.125ODHexBearing:4
- Mate:283: Intake Roller Plate:2 ↔ COTS_WCP-0783_1.125ODHexBearing:1
- Mate:284: Intake Roller Plate:2 ↔ COTS_217-2592_VersaHub:3
- Mate:285: Intake Roller Plate:2 ↔ COTS_217-2592_VersaHub:3
- Mate:286: Intake Roller Plate:2 ↔ COTS_217-2592_VersaHub:3
- Mate:287: Intake Roller Plate:2 ↔ COTS_WCP-0799_0.5inchHexShaftCollar:4
- Mate:288: COTS_WCP-0799_0.5inchHexShaftCollar:2 ↔ COTS_WCP-0799_0.5inchHexShaftCollar:4
- Mate:289: Intake BeaterBar:2 ↔ COTS_91251A539_Black-Oxide Alloy Steel Socket Head Screw (1):10
- Mate:290: Intake Roller Plate:2 ↔ Intake BeaterBar:2
- Mate:291: Intake Roller Plate:2 ↔ Intake BeaterBar:2
- Mate:292: Intake Roller Plate:2 ↔ COTS_91251A539_Black-Oxide Alloy Steel Socket Head Screw (1):10
- Mate:293: Intake Roller Plate:1 ↔ COTS_WCP-0783_1.125ODHexBearing:11
- Mate:294: Intake Roller Plate:1 ↔ COTS_WCP-0783_1.125ODHexBearing:10
- Mate:295: Intake Roller Plate:1 ↔ COTS_WCP-0783_1.125ODHexBearing:10
- Mate:296: Intake Roller Plate:1 ↔ COTS_91251A539_Black-Oxide Alloy Steel Socket Head Screw (1):2
- Mate:297: Intake Roller Plate:1 ↔ Intake BeaterBar:1
- Mate:298: Intake Roller Plate:1 ↔ Intake BeaterBar:1
- Mate:299: Intake Roller Plate:1 ↔ COTS_91251A539_Black-Oxide Alloy Steel Socket Head Screw (1):13
- Mate:300: Intake Roller Plate:2 ↔ COTS_91251A539_Black-Oxide Alloy Steel Socket Head Screw (1):9
- Mate:301: Intake Roller Plate:2 ↔ COTS_91251A539_Black-Oxide Alloy Steel Socket Head Screw (1):9
- Mate:302: Intake Roller Plate:1 ↔ COTS_217-2592_VersaHub:2
- Mate:303: Intake Roller Plate:1 ↔ COTS_217-2592_VersaHub:2
- Mate:304: Intake Roller Plate:1 ↔ COTS_217-2592_VersaHub:2
- Mate:305: COTS_217-2592_VersaHub:2 ↔ COTS_WCP-0799_0.5inchHexShaftCollar:1
- Mate:306: Intake Roller Plate:1 ↔ COTS_WCP-0799_0.5inchHexShaftCollar:1
- Mate:307: Intake Roller Plate:1 ↔ COTS_91251A539_Black-Oxide Alloy Steel Socket Head Screw (1):13
- Mate:308: Intake Roller Plate:1 ↔ COTS_REV-21-1650-V1.1:2
- Mate:310: Intake Roller Plate:1 ↔ COTS_REV-21-1650-V1.1:2
- Mate:311: Intake Roller Plate:1 ↔ COTS_REV-21-1650-V1.1:2
- Mate:312: Intake Roller Plate:1 ↔ Intake BeaterBar:2
- Mate:313: Intake Roller Plate:1 ↔ COTS_WCP-0783_1.125ODHexBearing:12
- Mate:315: Intake Roller Plate:1 ↔ COTS_WCP-0783_1.125ODHexBearing:8
- Mate:316: Intake Roller Plate:1 ↔ COTS_WCP-0783_1.125ODHexBearing:8
- Mate:317: Intake Roller Plate:1 ↔ COTS_WCP-0783_1.125ODHexBearing:9
- Mate:318: Intake Roller Plate:1 ↔ COTS_WCP-0783_1.125ODHexBearing:9
- Mate:319: Intake Roller Plate:1 ↔ COTS_WCP-0783_1.125ODHexBearing:7
- Mate:320: Intake Roller Plate:1 ↔ COTS_WCP-0783_1.125ODHexBearing:7
- Mate:321: Intake Roller Plate:1 ↔ COTS_WCP-0783_1.125ODHexBearing:11
- Mate:322: COTS_91251A539_Black-Oxide Alloy Steel Socket Head Screw (1):4 ↔ COTS_90107A029_316 Stainless Steel Washer:7
- Mate:323: COTS_WCP-0783_1.125ODHexBearing:10 ↔ COTS_90107A029_316 Stainless Steel Washer:9
- Mate:324: COTS_WCP-0783_1.125ODHexBearing:8 ↔ COTS_90107A029_316 Stainless Steel Washer:4
- Mate:326: COTS_WCP-0783_1.125ODHexBearing:7 ↔ COTS_90107A029_316 Stainless Steel Washer:1
- Mate:327: COTS_WCP-0783_1.125ODHexBearing:12 ↔ COTS_90107A029_316 Stainless Steel Washer:6
- Mate:328: COTS_WCP-0783_1.125ODHexBearing:11 ↔ COTS_90107A029_316 Stainless Steel Washer:7
- Mate:329: COTS_WCP-0783_1.125ODHexBearing:1 ↔ COTS_90107A029_316 Stainless Steel Washer:8
- Mate:330: COTS_WCP-0783_1.125ODHexBearing:4 ↔ COTS_90107A029_316 Stainless Steel Washer:5
- Mate:331: COTS_WCP-0783_1.125ODHexBearing:6 ↔ COTS_90107A029_316 Stainless Steel Washer:10
- Mate:332: COTS_WCP-0783_1.125ODHexBearing:3 ↔ COTS_90107A029_316 Stainless Steel Washer:12
- Mate:333: COTS_WCP-0783_1.125ODHexBearing:5 ↔ COTS_90107A029_316 Stainless Steel Washer:3
- Mate:334: COTS_WCP-0783_1.125ODHexBearing:2 ↔ COTS_90107A029_316 Stainless Steel Washer:11
- Mate:340: COTS_WCP-0783_1.125ODHexBearing:1 ↔ Intake HexShaft 1:6
- Mate:347: Intake Roller Plate:2 ↔ COTS_WCP-0783_1.125ODHexBearing:13
- Mate:348: Intake Roller Plate:2 ↔ COTS_WCP-0783_1.125ODHexBearing:13
- Flush:8: COTS_REV-21-1650-V1.1:2 ↔ Intake Hex Shaft 3:1
- Flush:10: COTS_WCP-0783_1.125ODHexBearing:1 ↔ Intake HexShaft 1:6
- Mate:355: COTS_WCP-0783_1.125ODHexBearing:1 ↔ COTS_90107A029_316 Stainless Steel Washer:8
- Mate:369: COTS_REV-21-1650-V1.1:2 ↔ COTW_HTD5M10mm12T_WCP-0076:1
- Mate:370: COTS_WCP-0783_1.125ODHexBearing:9 ↔ COTS_HTD5M10mm36T_WCP-0990:1
- Mate:371: COTS_WCP-0783_1.125ODHexBearing:9 ↔ COTS_HTD5M10mm36T_WCP-0990:1
- Flush:14: COTW_HTD5M10mm12T_WCP-0076:1 ↔ COTS_HTD5M10mm36T_WCP-0990:1
- Mate:372: COTS_WCP-0783_1.125ODHexBearing:6 ↔ COTS_WCP-0706_30T:1
- Mate:373: COTS_WCP-0783_1.125ODHexBearing:13 ↔ COTS_WCP-0706_30T:2
- Mate:374: COTS_WCP-0783_1.125ODHexBearing:6 ↔ COTS_WCP-0706_30T:1
- Mate:375: COTS_91251A539_Black-Oxide Alloy Steel Socket Head Screw (1):3 ↔ Intake Hex Shaft 3:1
- Mate:376: COTS_WCP-0783_1.125ODHexBearing:13 ↔ COTS_WCP-0706_30T:2
- Mate:377: COTS_WCP-0706_30T:2 ↔ COTS_HTD5M10mm18T_WCP-0563:1
- Mate:378: COTS_WCP-0706_30T:2 ↔ COTS_HTD5M10mm18T_WCP-0563:1
- Mate:379: COTS_WCP-0783_1.125ODHexBearing:2 ↔ COTS_HTD5M10mm18T_WCP-0563:2
- Mate:389: COTS_HTD5M10mm18T_WCP-0563:1 ↔ COTS_WCP-0783_1.125ODHexBearing:17
- Mate:390: COTS_90107A029_316 Stainless Steel Washer:10 ↔ COTS_WCP-0783_1.125ODHexBearing:15
- Mate:392: COTS_90107A029_316 Stainless Steel Washer:11 ↔ COTS_WCP-0783_1.125ODHexBearing:16
- Mate:393: COTS_WCP-0783_1.125ODHexBearing:17 ↔ INTK_002_HexShaft4:2
- Flush:16: COTS_WCP-0783_1.125ODHexBearing:17 ↔ INTK_002_HexShaft4:2
- Mate:394: COTS_91251A539_Black-Oxide Alloy Steel Socket Head Screw (1):17 ↔ COTS_90107A029_316 Stainless Steel Washer:13
- Mate:395: COTS_91251A539_Black-Oxide Alloy Steel Socket Head Screw (1):17 ↔ COTS_90107A029_316 Stainless Steel Washer:13
- Mate:396: COTS_91251A539_Black-Oxide Alloy Steel Socket Head Screw (1):18 ↔ COTS_90107A029_316 Stainless Steel Washer:14
- Mate:397: COTS_91251A539_Black-Oxide Alloy Steel Socket Head Screw (1):18 ↔ COTS_90107A029_316 Stainless Steel Washer:14
- Mate:398: INTK_002_HexShaft4:2 ↔ COTS_90107A029_316 Stainless Steel Washer:14
- Mate:399: INTK_002_HexShaft4:2 ↔ COTS_90107A029_316 Stainless Steel Washer:14
- Mate:400: INTK_002_HexShaft4:2 ↔ COTS_91251A539_Black-Oxide Alloy Steel Socket Head Screw (1):17
- Mate:401: INTK_002_HexShaft4:2 ↔ COTS_90107A029_316 Stainless Steel Washer:13
- Mate:402: COTS_WCP-0783_1.125ODHexBearing:11 ↔ INTK_003_HexShaft5:1
- Flush:17: COTS_WCP-0783_1.125ODHexBearing:11 ↔ INTK_003_HexShaft5:1
- Mate:403: COTS_WCP-0783_1.125ODHexBearing:11 ↔ COTS_90107A029_316 Stainless Steel Washer:7
- Mate:404: COTS_WCP-0783_1.125ODHexBearing:13 ↔ COTS_WCP-0783_1.125ODHexBearing:17
- Mate:405: COTS_WCP-0783_1.125ODHexBearing:6 ↔ COTS_WCP-0783_1.125ODHexBearing:15
- Mate:406: COTS_WCP-0783_1.125ODHexBearing:2 ↔ COTS_WCP-0783_1.125ODHexBearing:16
- Flush:19: COTS_WCP-0783_1.125ODHexBearing:16 ↔ INTK_003_HexShaft5:1
- Mate:407: COTS_WCP-0783_1.125ODHexBearing:9 ↔ Intake Hex Shaft 3:1
- Mate:408: COTS_91251A539_Black-Oxide Alloy Steel Socket Head Screw (1):3 ↔ COTS_90107A029_316 Stainless Steel Washer:2
- Mate:409: COTS_91251A539_Black-Oxide Alloy Steel Socket Head Screw (1):3 ↔ COTS_90107A029_316 Stainless Steel Washer:2
- Mate:410: Intake Hex Shaft 3:1 ↔ COTS_WCP-0783_1.125ODHexBearing:14
- Mate:414: COTS_90107A029_316 Stainless Steel Washer:2 ↔ COTS_WCP-0783_1.125ODHexBearing:14
- Mate:423: COTS_WCP-0783_1.125ODHexBearing:4 ↔ COTS_HTD5M10mm18T_WCP-0563:6
- Mate:425: COTS_WCP-0783_1.125ODHexBearing:10 ↔ COTS_HTD5M10mm18T_WCP-0563:5
- Flush:21: COTS_HTD5M10mm18T_WCP-0563:5 ↔ COTS_HTD5M10mm18T_WCP-0563:6
- Mate:426: COTS_91251A539_Black-Oxide Alloy Steel Socket Head Screw (1):15 ↔ COTS_90107A029_316 Stainless Steel Washer:5
- Mate:427: COTS_WCP-0783_1.125ODHexBearing:4 ↔ COTS_HTD5M10mm18T_WCP-0563:6
- Mate:428: COTS_WCP-0783_1.125ODHexBearing:1 ↔ COTS_WCP-0799_0.5inchHexShaftCollar:5
- Mate:429: COTS_HTD5M10mm18T_WCP-0563:5 ↔ COTS_WCP-0799_0.5inchHexShaftCollar:5
- Mate:430: COTS_WCP-0783_1.125ODHexBearing:4 ↔ COTS_WCP-0799_0.5inchHexShaftCollar:6
- Mate:431: COTS_HTD5M10mm18T_WCP-0563:6 ↔ COTS_WCP-0799_0.5inchHexShaftCollar:6
- Mate:432: COTS_WCP-0783_1.125ODHexBearing:10 ↔ COTS_HTD5M10mm18T_WCP-0563:18
- Mate:433: COTS_WCP-0783_1.125ODHexBearing:10 ↔ COTS_HTD5M10mm18T_WCP-0563:18
- Mate:434: COTS_WCP-0783_1.125ODHexBearing:8 ↔ COTS_HTD5M10mm18T_WCP-0563:16
- Mate:435: COTS_WCP-0783_1.125ODHexBearing:8 ↔ COTS_HTD5M10mm18T_WCP-0563:16
- Mate:436: COTS_HTD5M10mm18T_WCP-0563:18 ↔ COTS_WCP-0799_0.5inchHexShaftCollar:7
- Mate:437: COTS_HTD5M10mm18T_WCP-0563:18 ↔ COTS_WCP-0799_0.5inchHexShaftCollar:7
- Mate:438: COTS_HTD5M10mm18T_WCP-0563:16 ↔ COTS_WCP-0799_0.5inchHexShaftCollar:8
- Mate:439: COTS_HTD5M10mm18T_WCP-0563:16 ↔ COTS_WCP-0799_0.5inchHexShaftCollar:8
- Mate:440: COTS_WCP-0799_0.5inchHexShaftCollar:7 ↔ COTS_am-3462_2indiameter_0.500inhexbore_durometer35A_CompliantWheel:53
- Mate:441: COTS_WCP-0783_1.125ODHexBearing:7 ↔ COTS_am-3462_2indiameter_0.500inhexbore_durometer35A_CompliantWheel:25
- Mate:442: COTS_WCP-0783_1.125ODHexBearing:9 ↔ COTS_am-3462_2indiameter_0.500inhexbore_durometer35A_CompliantWheel:40
- Mate:443: COTS_WCP-0799_0.5inchHexShaftCollar:8 ↔ COTS_am-3462_2indiameter_0.500inhexbore_durometer35A_CompliantWheel:66
- Mate:444: COTS_WCP-0799_0.5inchHexShaftCollar:7 ↔ COTS_am-3462_2indiameter_0.500inhexbore_durometer35A_CompliantWheel:53
- Mate:445: COTS_WCP-0799_0.5inchHexShaftCollar:8 ↔ COTS_am-3462_2indiameter_0.500inhexbore_durometer35A_CompliantWheel:66
- Flush:22: COTS_am-3462_2indiameter_0.500inhexbore_durometer35A_CompliantWheel:66 ↔ COTS_am-3462_2indiameter_0.500inhexbore_durometer35A_CompliantWheel:40
- Flush:23: COTS_am-3462_2indiameter_0.500inhexbore_durometer35A_CompliantWheel:40 ↔ COTS_am-3462_2indiameter_0.500inhexbore_durometer35A_CompliantWheel:25
- Flush:24: COTS_am-3462_2indiameter_0.500inhexbore_durometer35A_CompliantWheel:25 ↔ COTS_am-3462_2indiameter_0.500inhexbore_durometer35A_CompliantWheel:24
- Mate:448: COTS_WCP-0783_1.125ODHexBearing:10 ↔ COTS_90107A029_316 Stainless Steel Washer:9
- Mate:454: COTS_90107A029_316 Stainless Steel Washer:4 ↔ INTK_004_HexShaft6:1
- Mate:455: COTS_WCP-0783_1.125ODHexBearing:7 ↔ COTS_HTD5M10mm18T_WCP-0563:4
- Mate:456: COTS_WCP-0783_1.125ODHexBearing:7 ↔ COTS_HTD5M10mm18T_WCP-0563:4
- Mate:457: COTS_91251A539_Black-Oxide Alloy Steel Socket Head Screw (1):14 ↔ COTS_HTD5M10mm18T_WCP-0563:12
- Mate:458: COTS_WCP-0783_1.125ODHexBearing:3 ↔ COTS_HTD5M10mm18T_WCP-0563:12
- Mate:459: COTS_91251A539_Black-Oxide Alloy Steel Socket Head Screw (1):14 ↔ COTS_WCP-0799_0.5inchHexShaftCollar:10
- Mate:460: COTS_HTD5M10mm18T_WCP-0563:12 ↔ COTS_WCP-0799_0.5inchHexShaftCollar:10
- Mate:461: COTS_HTD5M10mm18T_WCP-0563:4 ↔ COTS_WCP-0799_0.5inchHexShaftCollar:9
- Mate:462: COTS_HTD5M10mm18T_WCP-0563:4 ↔ COTS_WCP-0799_0.5inchHexShaftCollar:9
- Mate:463: COTS_WCP-0783_1.125ODHexBearing:9 ↔ COTS_HTD5M10mm18T_WCP-0563:14
- Mate:464: COTS_WCP-0783_1.125ODHexBearing:9 ↔ COTS_HTD5M10mm18T_WCP-0563:14
- Mate:465: COTS_HTD5M10mm18T_WCP-0563:14 ↔ COTS_WCP-0799_0.5inchHexShaftCollar:11
- Mate:466: COTS_HTD5M10mm18T_WCP-0563:14 ↔ COTS_WCP-0799_0.5inchHexShaftCollar:11
- Mate:467: COTS_WCP-0783_1.125ODHexBearing:6 ↔ COTS_WCP-0799_0.5inchHexShaftCollar:12
- Mate:468: COTS_WCP-0783_1.125ODHexBearing:6 ↔ COTS_HTD5M10mm18T_WCP-0563:9
- Mate:469: COTS_WCP-0783_1.125ODHexBearing:6 ↔ COTS_HTD5M10mm18T_WCP-0563:9
- Mate:470: COTS_HTD5M10mm18T_WCP-0563:9 ↔ COTS_WCP-0799_0.5inchHexShaftCollar:12
- Mate:472: COTS_90107A029_316 Stainless Steel Washer:4 ↔ COTS_WCP-0783_1.125ODHexBearing:19
- Mate:476: COTS_90107A029_316 Stainless Steel Washer:5 ↔ COTS_WCP-0783_1.125ODHexBearing:20
- Mate:479: COTS_WCP-0783_1.125ODHexBearing:5 ↔ COTS_HTD5M10mm18T_WCP-0563:11
- Mate:480: COTS_WCP-0783_1.125ODHexBearing:5 ↔ COTS_HTD5M10mm18T_WCP-0563:11
- Mate:481: Intake Roller Plate:1 ↔ COTS_WCP-0783_1.125ODHexBearing:12
- Mate:482: COTS_WCP-0783_1.125ODHexBearing:3 ↔ COTS_HTD5M10mm18T_WCP-0563:13
- Mate:483: COTS_WCP-0783_1.125ODHexBearing:12 ↔ COTS_HTD5M10mm18T_WCP-0563:15
- Mate:484: COTS_WCP-0783_1.125ODHexBearing:12 ↔ COTS_HTD5M10mm18T_WCP-0563:15
- Mate:485: COTS_WCP-0783_1.125ODHexBearing:7 ↔ COTS_HTD5M10mm18T_WCP-0563:17
- Flush:26: COTS_HTD5M10mm18T_WCP-0563:15 ↔ COTS_HTD5M10mm18T_WCP-0563:17
- Mate:496: COTS_90107A029_316 Stainless Steel Washer:3 ↔ COTS_WCP-0783_1.125ODHexBearing:24
- Mate:497: COTS_90107A029_316 Stainless Steel Washer:12 ↔ COTS_WCP-0783_1.125ODHexBearing:23
- Mate:498: COTS_90107A029_316 Stainless Steel Washer:6 ↔ COTS_WCP-0783_1.125ODHexBearing:21
- Mate:499: COTS_90107A029_316 Stainless Steel Washer:1 ↔ COTS_WCP-0783_1.125ODHexBearing:22
- Flush:29: COTS_HTD5M10mm18T_WCP-0563:1 ↔ COTS_HTD5M10mm18T_WCP-0563:2
- Mate:500: COTS_91251A539_Black-Oxide Alloy Steel Socket Head Screw (1):5 ↔ INTK_005_Spacer5:3
- Mate:501: COTS_WCP-0783_1.125ODHexBearing:2 ↔ INTK_005_Spacer5:3
- Mate:502: COTS_91251A539_Black-Oxide Alloy Steel Socket Head Screw (1):8 ↔ INTK_005_Spacer5:4
- Mate:503: COTS_HTD5M10mm18T_WCP-0563:11 ↔ INTK_005_Spacer5:4
- Mate:504: COTS_91251A539_Black-Oxide Alloy Steel Socket Head Screw (1):14 ↔ INTK_005_Spacer5:2
- Mate:505: COTS_WCP-0783_1.125ODHexBearing:23 ↔ INTK_005_Spacer5:2
- Mate:506: COTS_91251A539_Black-Oxide Alloy Steel Socket Head Screw (1):15 ↔ INTK_005_Spacer5:1
- Mate:508: COTS_WCP-0783_1.125ODHexBearing:8 ↔ INTK_005_Spacer5:5
- Mate:510: COTS_90107A029_316 Stainless Steel Washer:1 ↔ INTK_005_Spacer5:6
- Mate:511: COTS_HTD5M10mm18T_WCP-0563:17 ↔ INTK_005_Spacer5:6
- Mate:512: COTS_91251A539_Black-Oxide Alloy Steel Socket Head Screw (1):6 ↔ INTK_005_Spacer5:7
- Mate:513: COTS_WCP-0783_1.125ODHexBearing:21 ↔ INTK_005_Spacer5:7
- Mate:514: COTS_REV-21-1650-V1.1:2 ↔ INTK_006_Spacer6:1
- Flush:30: COTS_REV-21-1650-V1.1:2 ↔ INTK_006_Spacer6:1
- Mate:515: COTS_REV-21-1650-V1.1:2 ↔ COTS_91251A342_1-2in Long_Black-Oxide Alloy Steel Socket Head:3
- Mate:516: COTS_91251A342_1-2in Long_Black-Oxide Alloy Steel Socket Head:3 ↔ COTS_91860A047_Size10Washer:1
- Mate:517: COTS_91251A342_1-2in Long_Black-Oxide Alloy Steel Socket Head:3 ↔ COTS_91860A047_Size10Washer:1
- Mate:518: INTK_006_Spacer6:1 ↔ COTS_91860A047_Size10Washer:1
- Mate:520: Intake Roller Plate:1 ↔ COTS_91251A342_1-2in Long_Black-Oxide Alloy Steel Socket Head:1
- Mate:521: Intake Roller Plate:1 ↔ COTS_91251A342_1-2in Long_Black-Oxide Alloy Steel Socket Head:6
- Mate:525: Intake Roller Plate:1 ↔ COTS_91251A342_1-2in Long_Black-Oxide Alloy Steel Socket Head:6
- Mate:527: Intake Roller Plate:1 ↔ COTS_91251A342_1-2in Long_Black-Oxide Alloy Steel Socket Head:1
- Mate:529: COTS_WCP-0783_1.125ODHexBearing:4 ↔ INTK_005_Spacer5:1
- Mate:530: COTS_WCP-0706_30T:1 ↔ COTS_HTD5M10mm15T_WCP-1420:2
- Mate:531: COTS_WCP-0706_30T:1 ↔ COTS_HTD5M10mm15T_WCP-1420:2
- Mate:532: INTK_005_Spacer5:1 ↔ COTS_HTD5M10mm15T_WCP-1420:1
- Mate:533: INTK_005_Spacer5:1 ↔ COTS_HTD5M10mm15T_WCP-1420:1
- Mate:534: COTS_WCP-0783_1.125ODHexBearing:8 ↔ INTK_005_Spacer5:5
- Mate:535: COTS_HTD5M10mm36T_WCP-0990:1 ↔ COTS_HTD5M10mm15T_WCP-1420:4
- Mate:536: COTS_HTD5M10mm36T_WCP-0990:1 ↔ COTS_HTD5M10mm15T_WCP-1420:4
- Mate:537: COTS_WCP-0783_1.125ODHexBearing:19 ↔ COTS_HTD5M10mm15T_WCP-1420:3
- Mate:538: INTK_005_Spacer5:5 ↔ COTS_HTD5M10mm15T_WCP-1420:3
- Mate:539: COTS_WCP-0783_1.125ODHexBearing:19 ↔ COTS_HTD5M10mm15T_WCP-1420:3
- Flush:31: INTK_004_HexShaft6:3 ↔ COTS_WCP-0783_1.125ODHexBearing:22
- Mate:540: COTS_HTD5M10mm18T_WCP-0563:13 ↔ INTK_005_Spacer5:2
- Mate:541: COTS_WCP-0783_1.125ODHexBearing:3 ↔ COTS_HTD5M10mm18T_WCP-0563:13
- Mate:553: Intake Roller Plate:1 ↔ INTK_007_Spacer7:1
- Mate:555: Intake Roller Plate:1 ↔ INTK_007_Spacer7:8
- Mate:577: Intake Roller Plate:1 ↔ COTS_92949A265_1-2in long Stainless Steel Button Head Screw:6
- Mate:578: Intake Roller Plate:1 ↔ COTS_92949A265_1-2in long Stainless Steel Button Head Screw:20
- Mate:579: Intake Roller Plate:1 ↔ COTS_92949A265_1-2in long Stainless Steel Button Head Screw:8
- Mate:580: Intake Roller Plate:1 ↔ COTS_92949A265_1-2in long Stainless Steel Button Head Screw:19
- Mate:581: Intake Roller Plate:1 ↔ COTS_92949A265_1-2in long Stainless Steel Button Head Screw:21
- Mate:584: Intake Roller Plate:1 ↔ COTS_92949A265_1-2in long Stainless Steel Button Head Screw:21
- Mate:585: Intake Roller Plate:1 ↔ COTS_92949A265_1-2in long Stainless Steel Button Head Screw:19
- Mate:586: Intake Roller Plate:1 ↔ COTS_92949A265_1-2in long Stainless Steel Button Head Screw:6
- Mate:587: Intake Roller Plate:1 ↔ COTS_92949A265_1-2in long Stainless Steel Button Head Screw:20
- Mate:588: Intake Roller Plate:1 ↔ COTS_92949A265_1-2in long Stainless Steel Button Head Screw:8
- Mate:611: Intake Roller Plate:2 ↔ COTS_92949A265_1-2in long Stainless Steel Button Head Screw:11
- Mate:612: Intake Roller Plate:2 ↔ COTS_92949A265_1-2in long Stainless Steel Button Head Screw:25
- Mate:613: Intake Roller Plate:2 ↔ COTS_92949A265_1-2in long Stainless Steel Button Head Screw:27
- Mate:614: Intake Roller Plate:2 ↔ COTS_92949A265_1-2in long Stainless Steel Button Head Screw:23
- Mate:615: Intake Roller Plate:2 ↔ COTS_92949A265_1-2in long Stainless Steel Button Head Screw:22
- Mate:617: Intake Roller Plate:2 ↔ COTS_92949A265_1-2in long Stainless Steel Button Head Screw:22
- Mate:618: Intake Roller Plate:2 ↔ COTS_92949A265_1-2in long Stainless Steel Button Head Screw:23
- Mate:619: Intake Roller Plate:2 ↔ COTS_92949A265_1-2in long Stainless Steel Button Head Screw:27
- Mate:620: Intake Roller Plate:2 ↔ COTS_92949A265_1-2in long Stainless Steel Button Head Screw:25
- Mate:621: Intake Roller Plate:2 ↔ COTS_92949A265_1-2in long Stainless Steel Button Head Screw:11
- Mate:622: COTS_217-2592_VersaHub:2 ↔ COTS_91251A196_Black-Oxide Alloy Steel Socket Head Screw_5-8in:3
- Mate:623: COTS_217-2592_VersaHub:2 ↔ COTS_91251A196_Black-Oxide Alloy Steel Socket Head Screw_5-8in:1
- Mate:624: COTS_217-2592_VersaHub:2 ↔ COTS_91251A196_Black-Oxide Alloy Steel Socket Head Screw_5-8in:2
- Mate:625: COTS_217-2592_VersaHub:2 ↔ COTS_91251A196_Black-Oxide Alloy Steel Socket Head Screw_5-8in:11
- Mate:626: COTS_217-2592_VersaHub:2 ↔ COTS_91251A196_Black-Oxide Alloy Steel Socket Head Screw_5-8in:4
- Mate:627: COTS_217-2592_VersaHub:2 ↔ COTS_91251A196_Black-Oxide Alloy Steel Socket Head Screw_5-8in:6
- Mate:628: COTS_217-2592_VersaHub:2 ↔ COTS_91251A196_Black-Oxide Alloy Steel Socket Head Screw_5-8in:4
- Mate:629: COTS_217-2592_VersaHub:2 ↔ COTS_91251A196_Black-Oxide Alloy Steel Socket Head Screw_5-8in:6
- Mate:630: COTS_217-2592_VersaHub:2 ↔ COTS_91251A196_Black-Oxide Alloy Steel Socket Head Screw_5-8in:11
- Mate:631: COTS_217-2592_VersaHub:2 ↔ COTS_91251A196_Black-Oxide Alloy Steel Socket Head Screw_5-8in:2
- Mate:632: COTS_217-2592_VersaHub:2 ↔ COTS_91251A196_Black-Oxide Alloy Steel Socket Head Screw_5-8in:3
- Mate:633: COTS_217-2592_VersaHub:2 ↔ COTS_91251A196_Black-Oxide Alloy Steel Socket Head Screw_5-8in:1
- Mate:634: COTS_217-2592_VersaHub:3 ↔ COTS_91251A196_Black-Oxide Alloy Steel Socket Head Screw_5-8in:12
- Mate:635: COTS_217-2592_VersaHub:3 ↔ COTS_91251A196_Black-Oxide Alloy Steel Socket Head Screw_5-8in:7
- Mate:636: COTS_217-2592_VersaHub:3 ↔ COTS_91251A196_Black-Oxide Alloy Steel Socket Head Screw_5-8in:10
- Mate:637: COTS_217-2592_VersaHub:3 ↔ COTS_91251A196_Black-Oxide Alloy Steel Socket Head Screw_5-8in:9
- Mate:638: COTS_217-2592_VersaHub:3 ↔ COTS_91251A196_Black-Oxide Alloy Steel Socket Head Screw_5-8in:5
- Mate:639: COTS_217-2592_VersaHub:3 ↔ COTS_91251A196_Black-Oxide Alloy Steel Socket Head Screw_5-8in:8
- Mate:640: COTS_217-2592_VersaHub:3 ↔ COTS_91251A196_Black-Oxide Alloy Steel Socket Head Screw_5-8in:12
- Mate:641: COTS_217-2592_VersaHub:3 ↔ COTS_91251A196_Black-Oxide Alloy Steel Socket Head Screw_5-8in:7
- Mate:642: COTS_217-2592_VersaHub:3 ↔ COTS_91251A196_Black-Oxide Alloy Steel Socket Head Screw_5-8in:10
- Mate:643: COTS_217-2592_VersaHub:3 ↔ COTS_91251A196_Black-Oxide Alloy Steel Socket Head Screw_5-8in:8
- Mate:644: COTS_217-2592_VersaHub:3 ↔ COTS_91251A196_Black-Oxide Alloy Steel Socket Head Screw_5-8in:5